# Autodesk Inventor assembly: Bot 1
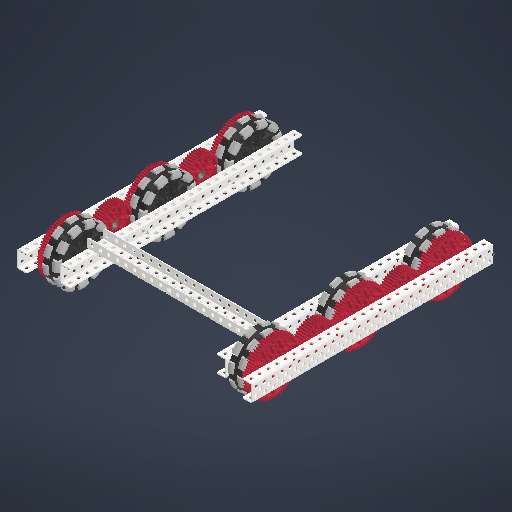
[picture p0: Inventor's stored thumbnail of the model, 512x512]
Saved by Autodesk Inventor 2025.2 (Build 292293000, 293)
## iProperties
Created: 2025-03-17
Part Number: Bot 1
Document SubType Name: Assembly
Designer: Jahan
Author: Jahan
## Documents named in this file (9)
- C:\1629X-7700R-Worlds-Bot\Bot 1\Bot 1.iam
- C:\1629X-7700R-Worlds-Bot\VEX-CAD-Inventor-1.4.2\Structure\C Channel\Aluminum 1x2x1\Alu C 1x2x1x27.ipt
- C:\1629X-7700R-Worlds-Bot\VEX-CAD-Inventor-1.4.2\Structure\C Channel\Aluminum 1x2x1\Alu C 1x2x1x19.ipt
- C:\1629X-7700R-Worlds-Bot\VEX-CAD-Inventor-1.4.2\Structure\C Channel\Aluminum 1x2x1\Alu C 1x2x1x28.ipt
- C:\1629X-7700R-Worlds-Bot\VEX-CAD-Inventor-1.4.2\Motion\Gears\HS Gear\HS 72T Gear, Circle.iam
- C:\1629X-7700R-Worlds-Bot\VEX-CAD-Inventor-1.4.2\Motion\Gears\HS Gear.iam
- C:\1629X-7700R-Worlds-Bot\VEX-CAD-Inventor-1.4.2\Motion\Wheels\Omni Wheel\3.25 Omni AS, No Insert.iam
- C:\1629X-7700R-Worlds-Bot\VEX-CAD-Inventor-1.4.2\Motion\Wheels\Omni Wheel.iam
- C:\1629X-7700R-Worlds-Bot\VEX-CAD-Inventor-1.4.2\Motion\Gears\HS Gear\HS 48T Gear, No Insert.iam
## Components (22 placed, 6 different names)
1. Alu C 1x2x1x19:1 — Insert:1, Insert:2, Insert:3, Insert:4
2. Alu C 1x2x1x27:1 — Insert:3, Insert:4
3. Alu C 1x2x1x27:2 — Insert:1, Insert:2, Insert:5, Insert:6
4. Alu C 1x2x1x27:3 — Insert:5, Insert:6, Insert:7, Insert:8, Insert:9, Insert:10
5. Alu C 1x2x1x28:1 — Insert:7, Insert:8, Insert:13, Insert:18, Insert:22, Insert:23, Insert:24
6. Alu C 1x2x1x28:2 — Insert:9, Insert:10, Insert:19, Insert:20, Insert:21, Insert:25, Insert:26
7. HS 72T Gear, Circle:1 [sub-assembly] — Insert:11, Insert:22
8. 3.25 Omni AS, No Insert:1 [sub-assembly] — Insert:11
9. HS 72T Gear, Circle:2 [sub-assembly] — Insert:13
10. 3.25 Omni AS, No Insert:2 [sub-assembly]
11. HS 72T Gear, Circle:3 [sub-assembly] — Insert:20
12. 3.25 Omni AS, No Insert:3 [sub-assembly]
13. HS 72T Gear, Circle:4 [sub-assembly] — Insert:19
14. 3.25 Omni AS, No Insert:4 [sub-assembly]
15. HS 72T Gear, Circle:5 [sub-assembly] — Insert:21
16. 3.25 Omni AS, No Insert:5 [sub-assembly]
17. HS 72T Gear, Circle:6 [sub-assembly] — Insert:18
18. 3.25 Omni AS, No Insert:6 [sub-assembly]
19. HS 48T Gear, No Insert:7 [sub-assembly] — Insert:23
20. HS 48T Gear, No Insert:8 [sub-assembly] — Insert:24
21. HS 48T Gear, No Insert:9 [sub-assembly] — Insert:25
22. HS 48T Gear, No Insert:10 [sub-assembly] — Insert:26
## Relationships (26: Insert 26)
- Insert:1: Alu C 1x2x1x19:1 ↔ Alu C 1x2x1x27:2
- Insert:2: Alu C 1x2x1x19:1 ↔ Alu C 1x2x1x27:2
- Insert:3: Alu C 1x2x1x19:1 ↔ Alu C 1x2x1x27:1
- Insert:4: Alu C 1x2x1x19:1 ↔ Alu C 1x2x1x27:1
- Insert:5: Alu C 1x2x1x27:2 ↔ Alu C 1x2x1x27:3
- Insert:6: Alu C 1x2x1x27:2 ↔ Alu C 1x2x1x27:3
- Insert:7: Alu C 1x2x1x27:3 ↔ Alu C 1x2x1x28:1
- Insert:8: Alu C 1x2x1x27:3 ↔ Alu C 1x2x1x28:1
- Insert:9: Alu C 1x2x1x27:3 ↔ Alu C 1x2x1x28:2
- Insert:10: Alu C 1x2x1x27:3 ↔ Alu C 1x2x1x28:2
- Insert:11: HS 72T Gear, Circle:1 ↔ 3.25 Omni AS, No Insert:1
- [Insert]: HS 72T Gear, Circle:2 ↔ 3.25 Omni AS, No Insert:2
- Insert:13 (15.875 mm): Alu C 1x2x1x28:1 ↔ HS 72T Gear, Circle:2
- [Insert]: HS 72T Gear, Circle:3 ↔ 3.25 Omni AS, No Insert:3
- [Insert]: HS 72T Gear, Circle:4 ↔ 3.25 Omni AS, No Insert:4
- [Insert]: HS 72T Gear, Circle:5 ↔ 3.25 Omni AS, No Insert:5
- [Insert]: HS 72T Gear, Circle:6 ↔ 3.25 Omni AS, No Insert:6
- Insert:18 (15.24 mm): Alu C 1x2x1x28:1 ↔ HS 72T Gear, Circle:6
- Insert:19 (15.875 mm): Alu C 1x2x1x28:2 ↔ HS 72T Gear, Circle:4
- Insert:20 (15.875 mm): Alu C 1x2x1x28:2 ↔ HS 72T Gear, Circle:3
- Insert:21 (15.875 mm): Alu C 1x2x1x28:2 ↔ HS 72T Gear, Circle:5
- Insert:22 (15.875 mm): Alu C 1x2x1x28:1 ↔ HS 72T Gear, Circle:1
- Insert:23 (15.875 mm): Alu C 1x2x1x28:1 ↔ HS 48T Gear, No Insert:7
- Insert:24 (15.875 mm): Alu C 1x2x1x28:1 ↔ HS 48T Gear, No Insert:8
- Insert:25 (15.875 mm): Alu C 1x2x1x28:2 ↔ HS 48T Gear, No Insert:9
- Insert:26 (15.875 mm): Alu C 1x2x1x28:2 ↔ HS 48T Gear, No Insert:10
## Named parameters: d91_d90 = 0 mm, d93_d90 = 0 mm, d94_d90 = 0 mm, d95_d90 = 0 mm, d96_d90 = 0 mm
